# Autodesk Inventor assembly: Сборка
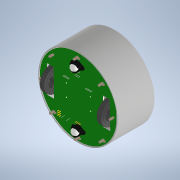
[picture p0: Inventor's stored thumbnail of the model, 180x180]
Saved by Autodesk Inventor 2020 (Build 240168000, 168)
## iProperties
Created: 2020-05-07
Part Number: Сборка
Document SubType Name: Assembly
Designer: jamnissa
Author: jamnissa
## Documents named in this file (11)
- C:\Users\jama1\Documents\GitHub\JRobots\pcbCase\Сборка.iam
- C:\Users\jama1\Documents\GitHub\JRobots\pcbCase\wheel\Wheel.ipt
- C:\Users\jama1\Documents\GitHub\JRobots\pcbCase\motor\motor.iam
- C:\Users\jama1\Documents\GitHub\JRobots\pcbCase\soporte_plastico\soporte_plastico.ipt
- C:\Users\jama1\Documents\GitHub\JRobots\pcbCase\Board\PcbBoard_last3.iam
- C:\Users\jama1\Documents\GitHub\JRobots\pcbCase\ball\ball.iam
- C:\Users\jama1\Documents\GitHub\JRobots\pcbCase\M3x6x25.ipt
- C:\Users\jama1\Documents\GitHub\JRobots\pcbCase\pcbCase\pcbCase_last.ipt
- C:\Users\jama1\Documents\GitHub\JRobots\pcbCase\case18650\case18650.ipt
- C:\Users\jama1\Documents\GitHub\JRobots\pcbCase\case18650\18650.ipt
- C:\Users\jama1\Documents\GitHub\JRobots\pcbCase\pcbCase\caseTop.ipt
## Components (22 placed, 10 different names)
1. Wheel:1 — ЗубчПер:1, Совмещение:6, Совмещение:12
2. Wheel:2 — Совмещение:7, Совмещение:13
3. motor:1 [sub-assembly] — Совмещение:7, Совмещение:13
4. motor:2 [sub-assembly] — ЗубчПер:1, Совмещение:6, Совмещение:12
5. soporte_plastico:1 — Совмещение:14
6. soporte_plastico:2
7. PcbBoard_last3:1 [sub-assembly] — Совмещение:14, Совмещение:15, Совмещение:16, Совмещение:17, Совмещение:18, Совмещение:19, Совмещение:20, Совмещение:22, Совмещение:23, Совмещение:24, Совмещение:25
8. ball:1 [sub-assembly] — Совмещение:15
9. ball:2 [sub-assembly] — Совмещение:16
10. M3x6x25:1 — Совмещение:17
11. M3x6x25:2 — Совмещение:25
12. M3x6x25:3 — Совмещение:19
13. M3x6x25:4 — Совмещение:20
14. M3x6x25:5 — Совмещение:24
15. M3x6x25:6 — Совмещение:22
16. M3x6x25:7 — Совмещение:23
17. M3x6x25:8 — Совмещение:18
18. pcbCase_last:1 — Совмещение:26
19. case18650:1 — Совмещение:26, Совмещение:27
20. 18650:1
21. 18650:2 — Совмещение:27
22. caseTop:1
## Relationships (18: Mate 17, RelateRotation 1)
- ЗубчПер:1 [RelateRotation] (1 ul): Wheel:1 ↔ motor:2
- Совмещение:6 [Mate]: Wheel:1 ↔ motor:2
- Совмещение:7 [Mate]: Wheel:2 ↔ motor:1
- Совмещение:12 [Mate]: Wheel:1 ↔ motor:2
- Совмещение:13 [Mate]: Wheel:2 ↔ motor:1
- Совмещение:14 [Mate]: soporte_plastico:1 ↔ PcbBoard_last3:1
- Совмещение:15 [Mate]: PcbBoard_last3:1 ↔ ball:1
- Совмещение:16 [Mate]: PcbBoard_last3:1 ↔ ball:2
- Совмещение:17 [Mate]: PcbBoard_last3:1 ↔ M3x6x25:1
- Совмещение:18 [Mate]: PcbBoard_last3:1 ↔ M3x6x25:8
- Совмещение:19 [Mate]: PcbBoard_last3:1 ↔ M3x6x25:3
- Совмещение:20 [Mate]: PcbBoard_last3:1 ↔ M3x6x25:4
- Совмещение:22 [Mate]: PcbBoard_last3:1 ↔ M3x6x25:6
- Совмещение:23 [Mate]: PcbBoard_last3:1 ↔ M3x6x25:7
- Совмещение:24 [Mate]: PcbBoard_last3:1 ↔ M3x6x25:5
- Совмещение:25 [Mate]: PcbBoard_last3:1 ↔ M3x6x25:2
- Совмещение:26 [Mate]: pcbCase_last:1 ↔ case18650:1
- Совмещение:27 [Mate]: case18650:1 ↔ 18650:2
